# Autodesk Inventor assembly: Filtro
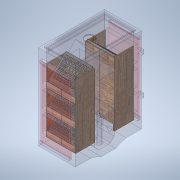
[picture p0: Inventor's stored thumbnail of the model, 180x180]
Saved by Autodesk Inventor 2021 (Build 250183000, 183)
## iProperties
Created: 2021-06-28
Part Number: Filtro
Document SubType Name: Assembly
Designer: artur
Mass: 25232.3 g
Surface Area: 23689.2 cm^2
Volume: 13297.3 cm^3
Density: 1.89755 g/cm^3
Author: artur
## Documents named in this file (16)
- C:\Users\artur\Downloads\Inventor\Filtro.iam
- C:\Users\artur\Downloads\Inventor\Contenedor.ipt
- C:\Users\artur\Downloads\Inventor\Interior Der.ipt
- C:\Users\artur\Downloads\Inventor\Interior Izq.ipt
- C:\Users\artur\Downloads\Inventor\Tornillo.ipt
- C:\Users\artur\Downloads\Inventor\Placa.ipt
- C:\Users\artur\Downloads\Inventor\Tapa.ipt
- C:\Users\artur\Downloads\Inventor\Rejilla_12x12mm.ipt
- C:\Users\artur\Downloads\Inventor\Rejilla_8x8mm.ipt
- C:\Users\artur\Downloads\Inventor\Rejilla_4x4mm.ipt
- C:\Users\artur\Downloads\Inventor\Filtro\AIP\FEA\dozqanakg.fins
- C:\Users\artur\Downloads\Inventor\Filtro\AIP\FEA\dozqanakg.fsat
- C:\Users\artur\Downloads\Inventor\Filtro\AIP\FEA\dozqanakg.ftes
- C:\Users\artur\Downloads\Inventor\Filtro\AIP\FEA\dozqanakg.fwiz
- C:\Users\artur\Downloads\Inventor\Filtro\AIP\FEA\dozqanav4.fmsh
- C:\Users\artur\Downloads\Inventor\Filtro\AIP\FEA\dozqanav5.fres
## Components (26 placed, 9 different names)
1. Contenedor:1 — Coincidencia:3, Coincidencia:4, Coincidencia:5, Coincidencia:6, Coincidencia:7, Coincidencia:8, Coincidencia:9, Coincidencia:10, Coincidencia:11, Coincidencia:12, Coincidencia:13, Coincidencia:14, Coincidencia:15, Coincidencia:16, Coincidencia:17
2. Interior Der:1 — Nivelación:1, Nivelación:2, Coincidencia:1, Coincidencia:29, Coincidencia:36, Coincidencia:37, Coincidencia:38, Coincidencia:39, Coincidencia:40, Coincidencia:41, Coincidencia:42, Coincidencia:43
3. Interior Izq:1 — Nivelación:1, Nivelación:2, Coincidencia:1, Coincidencia:3, Coincidencia:4, Insertar:1, Insertar:2, Insertar:3, Insertar:4, Insertar:5, Insertar:6, Coincidencia:7
4. Interior Der:2 — Nivelación:3, Nivelación:4, Coincidencia:2, Coincidencia:6, Coincidencia:20
5. Interior Izq:2 — Nivelación:3, Nivelación:4, Coincidencia:2, Coincidencia:5, Insertar:7, Insertar:8, Insertar:9, Insertar:10, Insertar:11, Insertar:12, Coincidencia:8, Coincidencia:19, Coincidencia:24, Coincidencia:30, Coincidencia:31, Coincidencia:32, Coincidencia:33, Coincidencia:34, Coincidencia:35
6. Tornillo:1 — Insertar:1
7. Tornillo:2 — Insertar:5
8. Tornillo:3 — Insertar:6
9. Tornillo:4 — Insertar:4
10. Tornillo:5 — Insertar:2
11. Tornillo:6 — Insertar:3
12. Tornillo:7 — Insertar:7
13. Tornillo:8 — Insertar:8
14. Tornillo:9 — Insertar:10
15. Tornillo:10 — Insertar:11
16. Tornillo:11 — Insertar:12
17. Tornillo:12 — Insertar:9
18. Placa:1 — Coincidencia:13, Coincidencia:14, Coincidencia:17
19. Placa:2 — Coincidencia:12, Coincidencia:15, Coincidencia:16
20. Tapa:1 — Coincidencia:9, Coincidencia:10, Coincidencia:11
21. Rejilla_12x12mm:2 — Coincidencia:29, Coincidencia:36, Coincidencia:37
22. Rejilla_8x8mm:1 — Coincidencia:20, Coincidencia:32, Coincidencia:33
23. Rejilla_8x8mm:2 — Coincidencia:38, Coincidencia:39, Coincidencia:40
24. Rejilla_4x4mm:1 — Coincidencia:24, Coincidencia:34, Coincidencia:35
25. Rejilla_4x4mm:2 — Coincidencia:41, Coincidencia:42, Coincidencia:43
26. Rejilla_12x12mm:3 — Coincidencia:19, Coincidencia:30, Coincidencia:31
## Relationships (51: Mate 35, Insert 12, Flush 4)
- Nivelación:1 [Flush]: Interior Der:1 ↔ Interior Izq:1
- Nivelación:2 [Flush]: Interior Der:1 ↔ Interior Izq:1
- Coincidencia:1 [Mate]: Interior Der:1 ↔ Interior Izq:1
- Nivelación:3 [Flush]: Interior Der:2 ↔ Interior Izq:2
- Nivelación:4 [Flush]: Interior Der:2 ↔ Interior Izq:2
- Coincidencia:2 [Mate]: Interior Der:2 ↔ Interior Izq:2
- Coincidencia:3 [Mate]: Contenedor:1 ↔ Interior Izq:1
- Coincidencia:4 [Mate]: Contenedor:1 ↔ Interior Izq:1
- Coincidencia:5 [Mate]: Contenedor:1 ↔ Interior Izq:2
- Coincidencia:6 [Mate]: Contenedor:1 ↔ Interior Der:2
- Insertar:1: Interior Izq:1 ↔ Tornillo:1
- Insertar:2: Interior Izq:1 ↔ Tornillo:5
- Insertar:3: Interior Izq:1 ↔ Tornillo:6
- Insertar:4: Interior Izq:1 ↔ Tornillo:4
- Insertar:5: Interior Izq:1 ↔ Tornillo:2
- Insertar:6: Interior Izq:1 ↔ Tornillo:3
- Coincidencia:7 [Mate]: Contenedor:1 ↔ Interior Izq:1
- Insertar:7: Interior Izq:2 ↔ Tornillo:7
- Insertar:8: Interior Izq:2 ↔ Tornillo:8
- Insertar:9: Interior Izq:2 ↔ Tornillo:12
- Insertar:10: Interior Izq:2 ↔ Tornillo:9
- Insertar:11: Interior Izq:2 ↔ Tornillo:10
- Insertar:12: Interior Izq:2 ↔ Tornillo:11
- Coincidencia:8 [Mate]: Contenedor:1 ↔ Interior Izq:2
- Coincidencia:9 [Mate]: Contenedor:1 ↔ Tapa:1
- Coincidencia:10 [Mate]: Contenedor:1 ↔ Tapa:1
- Coincidencia:11 [Mate]: Contenedor:1 ↔ Tapa:1
- Coincidencia:12 [Mate]: Contenedor:1 ↔ Placa:2
- Coincidencia:13 [Mate]: Contenedor:1 ↔ Placa:1
- Coincidencia:14 [Mate]: Contenedor:1 ↔ Placa:1
- Coincidencia:15 [Mate]: Contenedor:1 ↔ Placa:2
- Coincidencia:16 [Mate]: Contenedor:1 ↔ Placa:2
- Coincidencia:17 [Mate]: Contenedor:1 ↔ Placa:1
- Coincidencia:19 [Mate] (0.5 mm): Interior Izq:2 ↔ Rejilla_12x12mm:3
- Coincidencia:20 [Mate] (0.5 mm): Interior Der:2 ↔ Rejilla_8x8mm:1
- Coincidencia:24 [Mate] (0.5 mm): Interior Izq:2 ↔ Rejilla_4x4mm:1
- Coincidencia:29 [Mate] (0.5 mm): Interior Der:1 ↔ Rejilla_12x12mm:2
- Coincidencia:30 [Mate] (0.5 mm): Interior Izq:2 ↔ Rejilla_12x12mm:3
- Coincidencia:31 [Mate]: Interior Izq:2 ↔ Rejilla_12x12mm:3
- Coincidencia:32 [Mate] (0.5 mm): Interior Izq:2 ↔ Rejilla_8x8mm:1
- Coincidencia:33 [Mate]: Interior Izq:2 ↔ Rejilla_8x8mm:1
- Coincidencia:34 [Mate] (0.5 mm): Interior Izq:2 ↔ Rejilla_4x4mm:1
- Coincidencia:35 [Mate]: Interior Izq:2 ↔ Rejilla_4x4mm:1
- Coincidencia:36 [Mate] (0.5 mm): Interior Der:1 ↔ Rejilla_12x12mm:2
- Coincidencia:37 [Mate]: Interior Der:1 ↔ Rejilla_12x12mm:2
- Coincidencia:38 [Mate] (0.5 mm): Interior Der:1 ↔ Rejilla_8x8mm:2
- Coincidencia:39 [Mate] (0.5 mm): Interior Der:1 ↔ Rejilla_8x8mm:2
- Coincidencia:40 [Mate]: Interior Der:1 ↔ Rejilla_8x8mm:2
- Coincidencia:41 [Mate] (0.5 mm): Interior Der:1 ↔ Rejilla_4x4mm:2
- Coincidencia:42 [Mate] (0.5 mm): Interior Der:1 ↔ Rejilla_4x4mm:2
- Coincidencia:43 [Mate]: Interior Der:1 ↔ Rejilla_4x4mm:2
## Named parameters: sa_0 = 3333.3, sa_1 = 3333.3, sa_2 = 3333.3, sa_3 = 43000, sa_4 = 43000
note: some values were not read from the file. Shown as the stored number, unit unknown: "sa_0", "sa_1", "sa_2", "sa_3", "sa_4".
